# Autodesk Inventor assembly: main_assembly
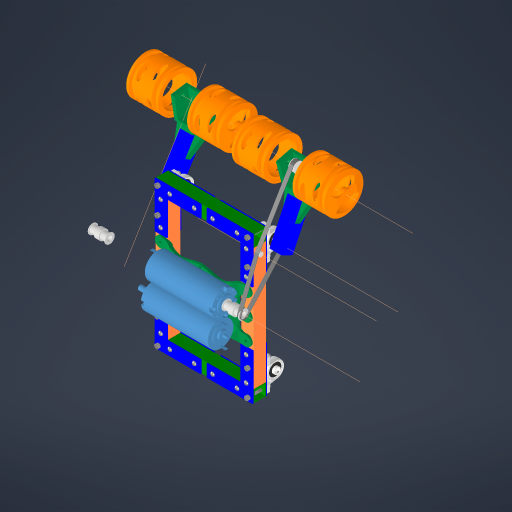
[picture p0: Inventor's stored thumbnail of the model, 512x512]
Saved by Autodesk Inventor 2024 (Build 280153000, 153)
## iProperties
Created: 2023-09-26
Part Number: main_assembly
Document SubType Name: Assembly
Designer: user
Author: user
## Documents named in this file (7)
- D:\Docs\Robot\3d_v2\main_assembly.iam
- D:\Docs\Robot\3d_v2\base\base_assambly.iam
- D:\Docs\Robot\3d_v2\machine_body\motor_holder_down.ipt
- D:\Docs\Robot\3d_v2\default_components\motor.ipt
- D:\Docs\Robot\3d_v2\default_components\double_gt2.ipt
- D:\Docs\Robot\3d_v2\machine_body\arm_assembly.iam
- D:\Docs\Robot\3d_v2\main_assembly\Мастер проектирования\Передача с помощью зубчатых ремней1.iam
## Components (9 placed, 6 different names)
1. base_assambly:1 [sub-assembly] — Совмещение:1, Совмещение:2, Совмещение:3, Совмещение:4, Совмещение:5, Совмещение:6, Совмещение:9, Угол:1, Угол:2, Вставка:2, Вставка:3
2. motor_holder_down:1 — Совмещение:4, Совмещение:5, Совмещение:6, Совмещение:7, Совмещение:8
3. motor:1 — Совмещение:7, Совмещение:9, Угол:1
4. motor:2 — Совмещение:8, Угол:2, Вставка:1
5. double_gt2:1 — Вставка:1
6. arm_assembly:1 [sub-assembly] — Вставка:2
7. arm_assembly:2 [sub-assembly] — Вставка:3, Совмещение:10, Совмещение:11
8. Передача с помощью зубчатых ремней:1 [sub-assembly]
9. double_gt2:2
## Relationships (16: Mate 11, Insert 3, Angle 2)
- Совмещение:1 [Mate]: base_assambly:1
- Совмещение:2 [Mate]: base_assambly:1
- Совмещение:3 [Mate]: base_assambly:1
- Совмещение:4 [Mate]: base_assambly:1 ↔ motor_holder_down:1
- Совмещение:5 [Mate]: base_assambly:1 ↔ motor_holder_down:1
- Совмещение:6 [Mate]: base_assambly:1 ↔ motor_holder_down:1
- Совмещение:7 [Mate]: motor_holder_down:1 ↔ motor:1
- Совмещение:8 [Mate]: motor_holder_down:1 ↔ motor:2
- Совмещение:9 [Mate]: base_assambly:1 ↔ motor:1
- Угол:1 [Angle] (90 deg): base_assambly:1 ↔ motor:1
- Угол:2 [Angle] (90 deg): base_assambly:1 ↔ motor:2
- Вставка:1 [Insert]: motor:2 ↔ double_gt2:1
- Вставка:2 [Insert]: base_assambly:1 ↔ arm_assembly:1
- Вставка:3 [Insert]: base_assambly:1 ↔ arm_assembly:2
- Совмещение:10 [Mate]: arm_assembly:2
- Совмещение:11 [Mate]: arm_assembly:2
